# Autodesk Inventor assembly: LR_04
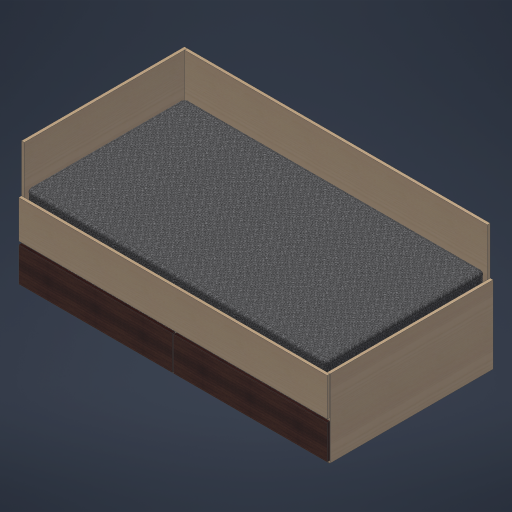
[picture p0: Inventor's stored thumbnail of the model, 512x512]
Saved by Autodesk Inventor 2024.3 (Build 283343000, 343)
## iProperties
Created: 2013-04-30
Part Number: LR_04
Document SubType Name: Assembly
Designer: SauliusD
Description: Bed
Material Code: Item.FillWorkpiece.Material.Code
Author: SauliusD
## Documents named in this file (26)
- C:\W4INV 2024 Design\PROJECTS\Living Room\Bed\LR_04.iam
- C:\W4INV 2024 Design\PROJECTS\Samples\Living Room\Bed\LR_0400.ipt
- C:\W4INV 2024 Design\PROJECTS\Samples\Living Room\Bed\LR_0406.ipt
- C:\W4INV 2024 Design\PROJECTS\Samples\Living Room\Bed\LR_0407.ipt
- C:\W4INV 2024 Design\PROJECTS\Samples\Living Room\Bed\LR_0415.ipt
- C:\W4INV 2024 Design\PROJECTS\Samples\Living Room\Bed\LR_0404.ipt
- C:\W4INV 2024 Design\PROJECTS\Samples\Living Room\Bed\LR_0411.ipt
- C:\W4INV 2024 Design\PROJECTS\Samples\Living Room\Bed\LR_0403.ipt
- C:\W4INV 2024 Design\PROJECTS\Samples\Living Room\Bed\LR_0410.ipt
- C:\W4INV 2024 Design\PROJECTS\Samples\Living Room\Bed\LR_0409.ipt
- C:\W4INV 2024 Design\PROJECTS\Samples\Living Room\Bed\LR_0402.ipt
- C:\W4INV 2024 Design\PROJECTS\Samples\Living Room\Bed\LR_0405.ipt
- C:\W4INV 2024 Design\PROJECTS\Samples\Living Room\Bed\LR_0408.ipt
- C:\W4INV 2024 Design\PROJECTS\Samples\Living Room\Bed\LR_0412.ipt
- C:\W4INV 2024 Design\PROJECTS\Samples\Living Room\Bed\LR_0413.ipt
- C:\W4INV 2024 Design\PROJECTS\Samples\Living Room\Bed\LR_0401.ipt
- C:\W4INV 2024 Design\PROJECTS\Samples\Living Room\Bed\LR_0416.ipt
- C:\W4INV 2024 Design\PROJECTS\Samples\Living Room\Bed\LR_0414.ipt
- C:\W4INV 2024 Design\_LIBRARY\Fixed joints\Confirmat\CONFIRMAT\Confirmat L50 & Cap D10 NB T18 PB T 18.ipt
- C:\W4INV 2023 Design\_LIBRARY\Fixed joints\Confirmat\CONFIRMAT\Confirmat L50 NB T18 PB T 18.ipt
- C:\W4INV 2024 Design\PROJECTS\Samples\Living Room\Bed\Drawer\BDR_Full Pull Drawer1.iam
- C:\W4INV 2024 Design\_LIBRARY\Fixed joints\Minifix joint\MINIFIX D15 v2\Minifix D15 & Dowel L34 & Cap D15 PB T18 LH.ipt
- C:\W4INV 2024 Design\_LIBRARY\Fixed joints\Minifix joint\MINIFIX D15 v2\Minifix D15 & Dowel L34 & Cap D15 PB T18 RH.ipt
- C:\W4INV 2023 Design\LIBRARY\Fixed joints\Confirmat\CONFIRMAT.ipt
- C:\W4INV 2023 Design\LIBRARY\Fixed joints\Minifix joint\MINIFIX D15 v2.ipt
- C:\W4INV 2023 Design\PROJECTS\Samples\Living Room\Bed\LR_04.iam
## Components (42 placed, 22 different names)
1. LR_0400-Mattress:1
2. LR_0406-Lattice:1
3. LR_0407-Allong Support:1
4. LR_0415-Short Lattice:1
5. LR_0404-Lattice End Support:1 — Mate:52, Flush:80, Flush:82, Mate:83, Mate:89
6. LR_0411-Lattice Front Support:1 — Flush:29, Flush:79, Flush:81, Mate:79, Mate:85
7. LR_0403-Lattice Facade Side Support:1 — Flush:78, Mate:74, Mate:76
8. LR_0410-Lattice Back Side Support:1 — Mate:70, Mate:72
9. LR_0409-Back Board:1 — Flush:75, Flush:76, Flush:77, Flush:95, Flush:96, Flush:97, Flush:98
10. LR_0402-Facade Board:1 — Flush:47, Mate:95, Mate:97, Mate:99, Mate:101
11. LR_0405-Bed-Head:1 — Flush:17, Flush:18, Mate:90, Mate:91, Mate:92, Flush:91, Flush:93, Mate:107, Mate:109
12. LR_0408-Foot:1 — Flush:21, Flush:92, Flush:94, Mate:103, Mate:105
13. LR_0413-Croos Support:1 — Flush:3, Flush:4, Flush:24, Mate:63, Mate:65, Mate:66, Mate:68, Mate:81, Mate:87, Mate:93, Flush:89
14. LR_0401-Bottom:1 — Mate:53, Flush:58
15. LR_0416-Lattice Middle Support:1 — Flush:33, Flush:34, Flush:83, Flush:84, Flush:85, Flush:86, Flush:87, Flush:88
16. LR_0412-Drawers Left Facade:1
17. LR_0414-Drawer Right Facade:1
18. LR_0401-Bottom:2 — Mate:52, Mate:53, Flush:58
19. Confirmat L50 & Cap D10 NB T18 PB T 18:2 — Mate:62, Flush:75, Mate:63
20. Confirmat L50 & Cap D10 NB T18 PB T 18:3 — Mate:64, Flush:76, Mate:65
21. Confirmat L50 & Cap D10 NB T18 PB T 18:4 — Flush:77, Mate:66, Mate:67
22. Confirmat L50 NB T18 PB T 18:6 — Flush:78, Mate:68, Mate:69
23. Confirmat L50 NB T18 PB T 18:7 — Mate:70, Flush:79, Mate:71
24. Confirmat L50 & Cap D10 NB T18 PB T 18:8 — Mate:72, Flush:80, Mate:73
25. Confirmat L50 NB T18 PB T 18:9 — Mate:74, Flush:81, Mate:75
26. Confirmat L50 NB T18 PB T 18:10 — Mate:76, Flush:82, Mate:77
27. Confirmat L50 & Cap D10 NB T18 PB T 18:11 — Mate:78, Mate:79, Flush:83
28. Confirmat L50 & Cap D10 NB T18 PB T 18:12 — Mate:80, Mate:81, Flush:84
29. Confirmat L50 & Cap D10 NB T18 PB T 18:13 — Mate:82, Mate:83, Flush:85
30. Confirmat L50 & Cap D10 NB T18 PB T 18:14 — Mate:84, Mate:85, Flush:86
31. Confirmat L50 & Cap D10 NB T18 PB T 18:15 — Mate:86, Mate:87, Flush:87
32. Confirmat L50 & Cap D10 NB T18 PB T 18:16 — Mate:88, Mate:89, Flush:88
33. BDR_Full Pull Drawer1:2 [sub-assembly] — Mate:93, Flush:89, Flush:90
34. Minifix D15 & Dowel L34 & Cap D15 PB T18 RH:1 — Mate:94, Flush:91, Mate:95
35. Minifix D15 & Dowel L34 & Cap D15 PB T18 LH:2 — Mate:96, Flush:92, Mate:97
36. Minifix D15 & Dowel L34 & Cap D15 PB T18 LH:3 — Mate:98, Flush:93, Mate:99
37. Minifix D15 & Dowel L34 & Cap D15 PB T18 RH:4 — Mate:100, Flush:94, Mate:101
38. Minifix D15 & Dowel L34 & Cap D15 PB T18 LH:5 — Mate:102, Mate:103, Flush:95
39. Minifix D15 & Dowel L34 & Cap D15 PB T18 RH:6 — Mate:104, Mate:105, Flush:96
40. Minifix D15 & Dowel L34 & Cap D15 PB T18 RH:7 — Mate:106, Mate:107, Flush:97
41. Minifix D15 & Dowel L34 & Cap D15 PB T18 LH:8 — Mate:108, Mate:109, Flush:98
42. BDR_Full Pull Drawer1:1 [sub-assembly] — Mate:90, Mate:91, Mate:92, Flush:90
## Relationships (86: Mate 50, Flush 36)
- Flush:3 (-40 mm): LR_0413-Croos Support:1
- Flush:4 (-40 mm): LR_0413-Croos Support:1
- Flush:17 (-80 mm): LR_0405-Bed-Head:1
- Flush:18 (-100 mm): LR_0405-Bed-Head:1
- Flush:21 (-80 mm): LR_0408-Foot:1
- Flush:24 (-30 mm): LR_0413-Croos Support:1
- Flush:29 (-30 mm): LR_0411-Lattice Front Support:1
- Flush:33 (-20 mm): LR_0416-Lattice Middle Support:1
- Flush:34 (-20 mm): LR_0416-Lattice Middle Support:1
- Flush:47 (-40 mm): LR_0402-Facade Board:1
- Flush:50 (-100 mm)
- Mate:52: LR_0404-Lattice End Support:1 ↔ LR_0401-Bottom:2
- Mate:53: LR_0401-Bottom:1 ↔ LR_0401-Bottom:2
- Flush:58: LR_0401-Bottom:1 ↔ LR_0401-Bottom:2
- Mate:62: Confirmat L50 & Cap D10 NB T18 PB T 18:2
- Flush:75: LR_0409-Back Board:1 ↔ Confirmat L50 & Cap D10 NB T18 PB T 18:2
- Mate:63 (-9 mm): LR_0413-Croos Support:1 ↔ Confirmat L50 & Cap D10 NB T18 PB T 18:2
- Mate:64: Confirmat L50 & Cap D10 NB T18 PB T 18:3
- Flush:76: LR_0409-Back Board:1 ↔ Confirmat L50 & Cap D10 NB T18 PB T 18:3
- Mate:65 (-9 mm): LR_0413-Croos Support:1 ↔ Confirmat L50 & Cap D10 NB T18 PB T 18:3
- Flush:77: LR_0409-Back Board:1 ↔ Confirmat L50 & Cap D10 NB T18 PB T 18:4
- Mate:66 (-9 mm): LR_0413-Croos Support:1 ↔ Confirmat L50 & Cap D10 NB T18 PB T 18:4
- Mate:67: Confirmat L50 & Cap D10 NB T18 PB T 18:4
- Flush:78: LR_0403-Lattice Facade Side Support:1 ↔ Confirmat L50 NB T18 PB T 18:6
- Mate:68 (-9 mm): LR_0413-Croos Support:1 ↔ Confirmat L50 NB T18 PB T 18:6
- Mate:69: Confirmat L50 NB T18 PB T 18:6
- Mate:70 (-9 mm): LR_0410-Lattice Back Side Support:1 ↔ Confirmat L50 NB T18 PB T 18:7
- Flush:79: LR_0411-Lattice Front Support:1 ↔ Confirmat L50 NB T18 PB T 18:7
- Mate:71: Confirmat L50 NB T18 PB T 18:7
- Mate:72 (-9 mm): LR_0410-Lattice Back Side Support:1 ↔ Confirmat L50 & Cap D10 NB T18 PB T 18:8
- Flush:80: LR_0404-Lattice End Support:1 ↔ Confirmat L50 & Cap D10 NB T18 PB T 18:8
- Mate:73: Confirmat L50 & Cap D10 NB T18 PB T 18:8
- Mate:74 (-9 mm): LR_0403-Lattice Facade Side Support:1 ↔ Confirmat L50 NB T18 PB T 18:9
- Flush:81: LR_0411-Lattice Front Support:1 ↔ Confirmat L50 NB T18 PB T 18:9
- Mate:75: Confirmat L50 NB T18 PB T 18:9
- Mate:76 (-9 mm): LR_0403-Lattice Facade Side Support:1 ↔ Confirmat L50 NB T18 PB T 18:10
- Flush:82: LR_0404-Lattice End Support:1 ↔ Confirmat L50 NB T18 PB T 18:10
- Mate:77: Confirmat L50 NB T18 PB T 18:10
- Mate:78: Confirmat L50 & Cap D10 NB T18 PB T 18:11
- Mate:79 (-9 mm): LR_0411-Lattice Front Support:1 ↔ Confirmat L50 & Cap D10 NB T18 PB T 18:11
- Flush:83: LR_0416-Lattice Middle Support:1 ↔ Confirmat L50 & Cap D10 NB T18 PB T 18:11
- Mate:80: Confirmat L50 & Cap D10 NB T18 PB T 18:12
- Mate:81 (-9 mm): LR_0413-Croos Support:1 ↔ Confirmat L50 & Cap D10 NB T18 PB T 18:12
- Flush:84: LR_0416-Lattice Middle Support:1 ↔ Confirmat L50 & Cap D10 NB T18 PB T 18:12
- Mate:82: Confirmat L50 & Cap D10 NB T18 PB T 18:13
- Mate:83 (-9 mm): LR_0404-Lattice End Support:1 ↔ Confirmat L50 & Cap D10 NB T18 PB T 18:13
- Flush:85: LR_0416-Lattice Middle Support:1 ↔ Confirmat L50 & Cap D10 NB T18 PB T 18:13
- Mate:84: Confirmat L50 & Cap D10 NB T18 PB T 18:14
- Mate:85 (-9 mm): LR_0411-Lattice Front Support:1 ↔ Confirmat L50 & Cap D10 NB T18 PB T 18:14
- Flush:86: LR_0416-Lattice Middle Support:1 ↔ Confirmat L50 & Cap D10 NB T18 PB T 18:14
- Mate:86: Confirmat L50 & Cap D10 NB T18 PB T 18:15
- Mate:87 (-9 mm): LR_0413-Croos Support:1 ↔ Confirmat L50 & Cap D10 NB T18 PB T 18:15
- Flush:87: LR_0416-Lattice Middle Support:1 ↔ Confirmat L50 & Cap D10 NB T18 PB T 18:15
- Mate:88: Confirmat L50 & Cap D10 NB T18 PB T 18:16
- Mate:89 (-9 mm): LR_0404-Lattice End Support:1 ↔ Confirmat L50 & Cap D10 NB T18 PB T 18:16
- Flush:88: LR_0416-Lattice Middle Support:1 ↔ Confirmat L50 & Cap D10 NB T18 PB T 18:16
- Mate:90: LR_0405-Bed-Head:1 ↔ BDR_Full Pull Drawer1:1
- Mate:91: LR_0405-Bed-Head:1 ↔ BDR_Full Pull Drawer1:1
- Mate:92: LR_0405-Bed-Head:1 ↔ BDR_Full Pull Drawer1:1
- Mate:93: LR_0413-Croos Support:1 ↔ BDR_Full Pull Drawer1:2
- Flush:89: LR_0413-Croos Support:1 ↔ BDR_Full Pull Drawer1:2
- Flush:90: BDR_Full Pull Drawer1:2 ↔ BDR_Full Pull Drawer1:1
- Mate:94: Minifix D15 & Dowel L34 & Cap D15 PB T18 RH:1
- Flush:91 (18 mm): LR_0405-Bed-Head:1 ↔ Minifix D15 & Dowel L34 & Cap D15 PB T18 RH:1
- Mate:95: LR_0402-Facade Board:1 ↔ Minifix D15 & Dowel L34 & Cap D15 PB T18 RH:1
- Mate:96: Minifix D15 & Dowel L34 & Cap D15 PB T18 LH:2
- Flush:92 (18 mm): LR_0408-Foot:1 ↔ Minifix D15 & Dowel L34 & Cap D15 PB T18 LH:2
- Mate:97: LR_0402-Facade Board:1 ↔ Minifix D15 & Dowel L34 & Cap D15 PB T18 LH:2
- Mate:98: Minifix D15 & Dowel L34 & Cap D15 PB T18 LH:3
- Flush:93 (18 mm): LR_0405-Bed-Head:1 ↔ Minifix D15 & Dowel L34 & Cap D15 PB T18 LH:3
- Mate:99: LR_0402-Facade Board:1 ↔ Minifix D15 & Dowel L34 & Cap D15 PB T18 LH:3
- Mate:100: Minifix D15 & Dowel L34 & Cap D15 PB T18 RH:4
- Flush:94 (18 mm): LR_0408-Foot:1 ↔ Minifix D15 & Dowel L34 & Cap D15 PB T18 RH:4
- Mate:101: LR_0402-Facade Board:1 ↔ Minifix D15 & Dowel L34 & Cap D15 PB T18 RH:4
- Mate:102: Minifix D15 & Dowel L34 & Cap D15 PB T18 LH:5
- Mate:103: LR_0408-Foot:1 ↔ Minifix D15 & Dowel L34 & Cap D15 PB T18 LH:5
- Flush:95 (18 mm): LR_0409-Back Board:1 ↔ Minifix D15 & Dowel L34 & Cap D15 PB T18 LH:5
- Mate:104: Minifix D15 & Dowel L34 & Cap D15 PB T18 RH:6
- Mate:105: LR_0408-Foot:1 ↔ Minifix D15 & Dowel L34 & Cap D15 PB T18 RH:6
- Flush:96 (18 mm): LR_0409-Back Board:1 ↔ Minifix D15 & Dowel L34 & Cap D15 PB T18 RH:6
- Mate:106: Minifix D15 & Dowel L34 & Cap D15 PB T18 RH:7
- Mate:107: LR_0405-Bed-Head:1 ↔ Minifix D15 & Dowel L34 & Cap D15 PB T18 RH:7
- Flush:97 (18 mm): LR_0409-Back Board:1 ↔ Minifix D15 & Dowel L34 & Cap D15 PB T18 RH:7
- Mate:108: Minifix D15 & Dowel L34 & Cap D15 PB T18 LH:8
- Mate:109: LR_0405-Bed-Head:1 ↔ Minifix D15 & Dowel L34 & Cap D15 PB T18 LH:8
- Flush:98 (18 mm): LR_0409-Back Board:1 ↔ Minifix D15 & Dowel L34 & Cap D15 PB T18 LH:8
